# Autodesk Inventor assembly: ASDSAttachmentAssembly
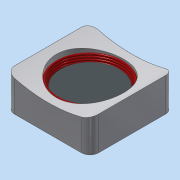
[picture p0: Inventor's stored thumbnail of the model, 180x180]
Saved by Autodesk Inventor 2017 (Build 210142000, 142)
## iProperties
Created: 2017-11-03
Part Number: ASDSAttachmentAssembly
Document SubType Name: Assembly
Designer: Derek Wider
Author: Derek Wider
## Documents named in this file (4)
- E:\OneDrive\Documents\Other Projects\Submarine\CAD\midships\ASDSAttachment\ASDSAttachmentAssembly.iam
- E:\OneDrive\Documents\Other Projects\Submarine\CAD\midships\ASDSAttachment\CoilHolder.ipt
- E:\OneDrive\Documents\Other Projects\Submarine\CAD\midships\ASDSAttachment\Coil.ipt
- E:\OneDrive\Documents\Other Projects\Submarine\CAD\midships\ASDSAttachment\FerriteCore.ipt
## Components (3 placed, 3 different names)
1. CoilHolder:1 — Mate:1, Mate:2, Mate:3, Flush:1
2. Coil:1 — Mate:1, Mate:2
3. FerriteCore:1 — Mate:3, Flush:1
## Relationships (4: Mate 3, Flush 1)
- Mate:1: CoilHolder:1 ↔ Coil:1
- Mate:2 (-0.889 mm): CoilHolder:1 ↔ Coil:1
- Mate:3: CoilHolder:1 ↔ FerriteCore:1
- Flush:1: CoilHolder:1 ↔ FerriteCore:1
